# Autodesk Inventor assembly: Return_Spool_Mount
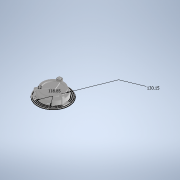
[picture p0: Inventor's stored thumbnail of the model, 180x180]
Saved by Autodesk Inventor 2022 (Build 260153070, 153G)
## iProperties
Created: 2022-03-05
Part Number: Return_Spool_Mount
Document SubType Name: Assembly
Designer: a laptop
Author: a laptop
## Documents named in this file (6)
- C:\Users\a laptop\Desktop\MDL_2021_Project\Return_Spool_Reel\Return_Spool_Mount.iam
- C:\Users\a laptop\Desktop\MDL_2021_Project\Return_Spool_Reel\Return_Spool_Mount.ipt
- C:\Users\a laptop\Desktop\MDL_2021_Project\Return_Spool_Reel\Return_Spool_Mount_2.ipt
- C:\Users\a laptop\Desktop\MDL_2021_Project\Return_Spool_Reel\Screws\M8 Washer98689A116_General Purpose 18-8 Stainless Steel Washer.ipt
- C:\Users\a laptop\Desktop\MDL_2021_Project\Return_Spool_Reel\Screws\92855A714_18-8 Stainless Steel Low-Profile Socket Head Screws.ipt
- C:\Users\a laptop\Desktop\MDL_2021_Project\Return_Spool_Reel\Return_Spool_Mount\Design Accelerator\Bearing2.iam
## Components (5 placed, 5 different names)
1. Return_Spool_Mount:1 — Mate:1, Mate:2, Mate:3
2. Return_Spool_Mount_2:1 — Mate:1, Mate:2, Mate:3, Mate:4, Mate:5, Mate:6, Mate:7
3. M8 Washer98689A116_General Purpose 18-8 Stainless Steel Washer:1 — Mate:4, Mate:5, Mate:8
4. 92855A714_18-8 Stainless Steel Low-Profile Socket Head Screws:1 — Mate:6, Mate:9
5. Bearing:1 [sub-assembly] — Mate:7, Mate:8, Mate:9
## Relationships (9: Mate 9)
- Mate:1: Return_Spool_Mount:1 ↔ Return_Spool_Mount_2:1
- Mate:2: Return_Spool_Mount:1 ↔ Return_Spool_Mount_2:1
- Mate:3: Return_Spool_Mount:1 ↔ Return_Spool_Mount_2:1
- Mate:4: Return_Spool_Mount_2:1 ↔ M8 Washer98689A116_General Purpose 18-8 Stainless Steel Washer:1
- Mate:5: Return_Spool_Mount_2:1 ↔ M8 Washer98689A116_General Purpose 18-8 Stainless Steel Washer:1
- Mate:6: Return_Spool_Mount_2:1 ↔ 92855A714_18-8 Stainless Steel Low-Profile Socket Head Screws:1
- Mate:7: Return_Spool_Mount_2:1 ↔ Bearing:1
- Mate:8: M8 Washer98689A116_General Purpose 18-8 Stainless Steel Washer:1 ↔ Bearing:1
- Mate:9: 92855A714_18-8 Stainless Steel Low-Profile Socket Head Screws:1 ↔ Bearing:1
